# Autodesk Inventor assembly: EccentricSpacerWheelAssembly
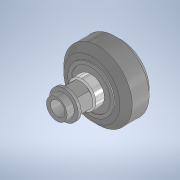
[picture p0: Inventor's stored thumbnail of the model, 180x180]
Saved by Autodesk Inventor 2022 (Build 260153000, 153)
## iProperties
Created: 2021-11-02
Part Number: EccentricSpacerWheelAssembly
Document SubType Name: Assembly
Designer: JK
Author: JK
## Documents named in this file (4)
- C:\Users\JK\Documents\Inventor\UTM\EccentricSpacerWheelAssembly.iam
- C:\Users\JK\Documents\Inventor\UTM\GantryPlateWheel.ipt
- C:\Users\JK\Documents\Inventor\UTM\EccentricSpacer.ipt
- C:\Users\JK\Documents\Inventor\UTM\3mmSpacer.ipt
## Components (3 placed, 3 different names)
1. GantryPlateWheel:1 — Coincidencia:2, Coincidencia:4
2. EccentricSpacer:1 — Coincidencia:3
3. 3mmSpacer:1 — Coincidencia:2, Coincidencia:3, Coincidencia:4
## Relationships (4: Mate 4)
- [Mate]: GantryPlateWheel:1 ↔ EccentricSpacer:1
- Coincidencia:2 [Mate]: GantryPlateWheel:1 ↔ 3mmSpacer:1
- Coincidencia:3 [Mate]: EccentricSpacer:1 ↔ 3mmSpacer:1
- Coincidencia:4 [Mate]: GantryPlateWheel:1 ↔ 3mmSpacer:1
